# Autodesk Inventor assembly: Сборка ручка
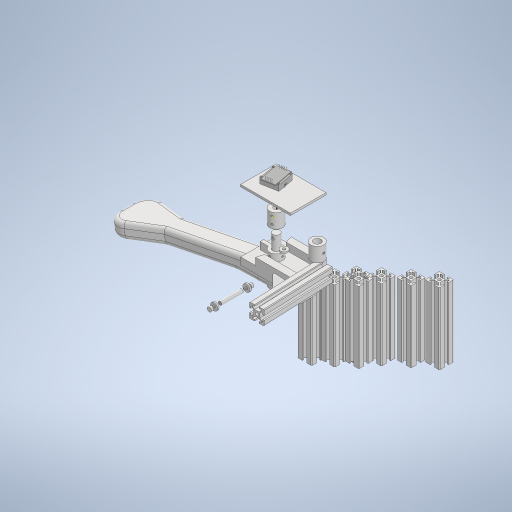
[picture p0: Inventor's stored thumbnail of the model, 512x512]
Saved by Autodesk Inventor 2023 (Build 270158000, 158)
## iProperties
Created: 2022-05-02
Part Number: Сборка ручка
Document SubType Name: Assembly
Designer: User
Author: User
## Documents named in this file (15)
- D:\Стойка\Механизм ручки\Сборка ручка.iam
- D:\Стойка\Механизм ручки\EAW.ipt
- D:\Стойка\Механизм ручки\Вал ручки.ipt
- D:\Стойка\Механизм ручки\Втулка энкодер.ipt
- D:\Стойка\Механизм ручки\Втулка.ipt
- D:\Стойка\Механизм ручки\Ручка.ipt
- D:\Стойка\Механизм ручки\Стенка.ipt
- D:\Стойка\Механизм ручки\Стопор.ipt
- D:\Стойка\Механизм ручки\Стенка энкодер.ipt
- D:\Стойка\Механизм ручки\Диск.ipt
- D:\Стойка\Механизм ручки\М3х8.ipt
- D:\Стойка\Механизм ручки\Шпилька.ipt
- D:\Стойка\Механизм ручки\Диск конец вала.ipt
- D:\Стойка\Механизм ручки\Балка 100 мм.ipt
- D:\Стойка\Механизм ручки\угол (1).ipt
## Components (25 placed, 14 different names)
1. EAW:1 — Цилиндрический:4
2. Вал ручки:1 — Цилиндрический:1, Совмещение:1, Цилиндрический:2, Цилиндрический:5, Совмещение:2, Цилиндрический:12
3. Втулка энкодер:1 — Цилиндрический:3, Цилиндрический:4
4. Втулка:1
5. Ручка:1 — Цилиндрический:1, Совмещение:1, Цилиндрический:6
6. Стенка:1 — Заподлицо:1, Заподлицо:2, Цилиндрический:5, Совмещение:3
7. Стопор:1 — Цилиндрический:2, Совмещение:2, Совмещение:3
8. Стенка энкодер:1 — Заподлицо:1, Цилиндрический:3, Заподлицо:2
9. Диск:1
10. М3х8:1 — Цилиндрический:11, Цилиндрический:12
11. Диск:2 — Цилиндрический:10
12. М3х8:2 — Цилиндрический:9, Цилиндрический:10
13. Диск:3 — Цилиндрический:8
14. М3х8:3 — Цилиндрический:7, Цилиндрический:8
15. Шпилька:1 — Цилиндрический:6, Цилиндрический:7, Цилиндрический:9
16. Диск конец вала:1 — Цилиндрический:11
17. Балка 100 мм:1
18. Балка 100 мм:2
19. Балка 100 мм:3
20. Балка 100 мм:4
21. Балка 100 мм:5
22. Балка 100 мм:6
23. Балка 100 мм:7
24. Балка 100 мм:8
25. угол (1):1
## Relationships (17: CylindricalJoint 12, Mate 3, Flush 2)
- Цилиндрический:1 [CylindricalJoint]: Вал ручки:1 ↔ Ручка:1
- Совмещение:1 [Mate]: Вал ручки:1 ↔ Ручка:1
- Цилиндрический:2 [CylindricalJoint]: Вал ручки:1 ↔ Стопор:1
- Заподлицо:1 [Flush]: Стенка:1 ↔ Стенка энкодер:1
- Цилиндрический:3 [CylindricalJoint]: Втулка энкодер:1 ↔ Стенка энкодер:1
- Цилиндрический:4 [CylindricalJoint]: EAW:1 ↔ Втулка энкодер:1
- Заподлицо:2 [Flush]: Стенка:1 ↔ Стенка энкодер:1
- Цилиндрический:5 [CylindricalJoint]: Вал ручки:1 ↔ Стенка:1
- Совмещение:2 [Mate]: Вал ручки:1 ↔ Стопор:1
- Совмещение:3 [Mate]: Стенка:1 ↔ Стопор:1
- Цилиндрический:6 [CylindricalJoint]: Ручка:1 ↔ Шпилька:1
- Цилиндрический:7 [CylindricalJoint]: М3х8:3 ↔ Шпилька:1
- Цилиндрический:8 [CylindricalJoint]: Диск:3 ↔ М3х8:3
- Цилиндрический:9 [CylindricalJoint]: М3х8:2 ↔ Шпилька:1
- Цилиндрический:10 [CylindricalJoint]: Диск:2 ↔ М3х8:2
- Цилиндрический:11 [CylindricalJoint]: М3х8:1 ↔ Диск конец вала:1
- Цилиндрический:12 [CylindricalJoint]: Вал ручки:1 ↔ М3х8:1
